# Autodesk Inventor assembly: 상단부 헤드 조립품
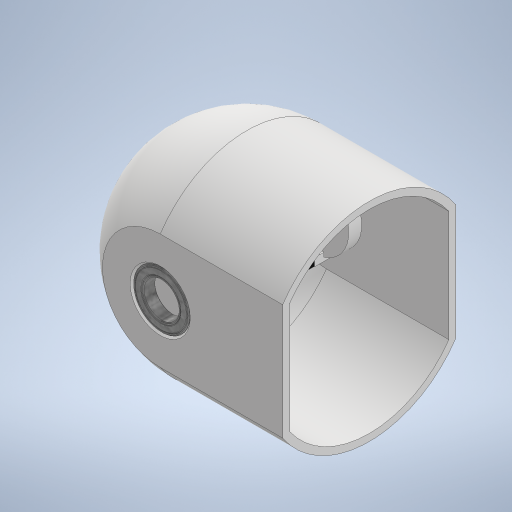
[picture p0: Inventor's stored thumbnail of the model, 512x512]
Saved by Autodesk Inventor 2023 (Build 270158000, 158)
## iProperties
Created: 2022-06-08
Part Number: 상단부 헤드 조립품
Document SubType Name: Assembly
Designer: fly01
Author: fly01
## Documents named in this file (6)
- C:\Users\fly01\Desktop\2022카이스트 입학준비\스마트홈\제작부품'\상단부 헤드 조립품.iam
- C:\Users\fly01\Desktop\2022카이스트 입학준비\스마트홈\범용 부품\6203베어링.ipt
- C:\Users\fly01\Desktop\2022카이스트 입학준비\스마트홈\제작부품'\메인 형상_상단 헤드.ipt
- C:\Users\fly01\Desktop\2022카이스트 입학준비\스마트홈\범용 부품\부속부품 2. 180도 서보모터.ipt
- C:\Users\fly01\Desktop\2022카이스트 입학준비\스마트홈\범용 부품\180도 서보모터 십자축 자른 것.ipt
- C:\Users\fly01\Desktop\2022카이스트 입학준비\스마트홈\범용 부품\십자 둥근머리 볼트 6mm.ipt
## Components (7 placed, 5 different names)
1. 메인 형상_상단 헤드:1 — 회전:1, 삽입:1, 삽입:2, 회전:2
2. 6203베어링:1 — 회전:1
3. 부속부품 2. 180도 서보모터:1 — 삽입:1, 삽입:2, 삽입:3, 강체:1, 강체:2
4. 180도 서보모터 십자축 자른 것:1 — 삽입:3
5. 십자 둥근머리 볼트 6mm:1 — 강체:1
6. 십자 둥근머리 볼트 6mm:2 — 강체:2
7. 6203베어링:2 — 회전:2
## Relationships (7: Insert 3, RevoluteJoint 2, WeldJoint 2)
- 회전:1 [RevoluteJoint]: 메인 형상_상단 헤드:1 ↔ 6203베어링:1
- 삽입:1 [Insert]: 메인 형상_상단 헤드:1 ↔ 부속부품 2. 180도 서보모터:1
- 삽입:2 [Insert]: 메인 형상_상단 헤드:1 ↔ 부속부품 2. 180도 서보모터:1
- 삽입:3 [Insert]: 부속부품 2. 180도 서보모터:1 ↔ 180도 서보모터 십자축 자른 것:1
- 강체:1 [WeldJoint]: 부속부품 2. 180도 서보모터:1 ↔ 십자 둥근머리 볼트 6mm:1
- 강체:2 [WeldJoint]: 부속부품 2. 180도 서보모터:1 ↔ 십자 둥근머리 볼트 6mm:2
- 회전:2 [RevoluteJoint]: 메인 형상_상단 헤드:1 ↔ 6203베어링:2
